# Autodesk Inventor assembly: PinecilCaseASM
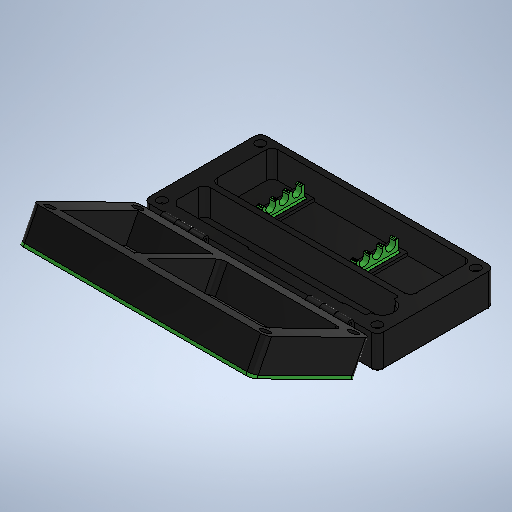
[picture p0: Inventor's stored thumbnail of the model, 512x512]
Saved by Autodesk Inventor 2026 (Build 300175050, 175E)
## iProperties
Created: 2025-10-09
Part Number: PinecilCaseASM
Document SubType Name: Assembly
Designer: Nicholas M
Author: Nicholas M
## Documents named in this file (6)
- C:\Users\nmari\OneDrive\Documents\Inventor Parts\pinecil-case\PinecilCaseASM.iam
- C:\Users\nmari\OneDrive\Documents\Inventor Parts\pinecil-case\PinecilCaseBottom.ipt
- C:\Users\nmari\OneDrive\Documents\Inventor Parts\pinecil-case\Pinecil Clip.ipt
- C:\Users\nmari\OneDrive\Documents\Inventor Parts\pinecil-case\PinecilCaseTop.ipt
- C:\Users\nmari\OneDrive\Documents\Inventor Parts\pinecil-case\PinecilLogo.ipt
- C:\Users\nmari\OneDrive\Documents\Inventor Parts\pinecil-case\PinecilCaseBorder.ipt
## Components (6 placed, 5 different names)
1. PinecilCaseBottom:1 — Mate:2, Mate:3, Angle:1, Rigid:5, Rigid:6
2. Pinecil Clip:1 — Rigid:6
3. Pinecil Clip:2 — Rigid:5
4. PinecilCaseTop:1 — Mate:2, Mate:3, Angle:1, Rigid:3, Mate:4, Flush:1, Flush:2
5. PinecilLogo:1 — Rigid:3
6. PinecilCaseBorder:1 — Mate:4, Flush:1, Flush:2
## Relationships (9: Mate 3, WeldJoint 3, Flush 2, Angle 1)
- Mate:2 (0.127 mm): PinecilCaseBottom:1 ↔ PinecilCaseTop:1
- Mate:3: PinecilCaseBottom:1 ↔ PinecilCaseTop:1
- Angle:1 (0 deg): PinecilCaseBottom:1 ↔ PinecilCaseTop:1
- Rigid:3 [WeldJoint]: PinecilCaseTop:1 ↔ PinecilLogo:1
- Rigid:5 [WeldJoint]: PinecilCaseBottom:1 ↔ Pinecil Clip:2
- Rigid:6 [WeldJoint]: PinecilCaseBottom:1 ↔ Pinecil Clip:1
- Mate:4: PinecilCaseTop:1 ↔ PinecilCaseBorder:1
- Flush:1: PinecilCaseTop:1 ↔ PinecilCaseBorder:1
- Flush:2: PinecilCaseTop:1 ↔ PinecilCaseBorder:1
